# Autodesk Inventor assembly: LockMechanism_v3
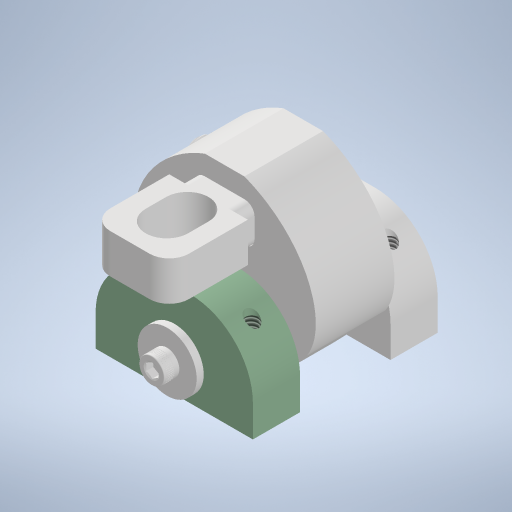
[picture p0: Inventor's stored thumbnail of the model, 512x512]
Saved by Autodesk Inventor 2023 (Build 270158000, 158)
## iProperties
Created: 2023-01-14
Part Number: LockMechanism_v3
Document SubType Name: Assembly
Designer: Hayden Swanson
Author: Hayden Swanson
## Documents named in this file (8)
- C:\Users\Hayden Swanson\UNLAssemblyProject\Hardware\ETL\Module Assembly\WAM_v3\LockMechanism_v3.iam
- C:\Users\Hayden Swanson\UNLAssemblyProject\Hardware\ETL\Module Assembly\WAM_v3\cam3.ipt
- C:\Users\Hayden Swanson\UNLAssemblyProject\Hardware\ETL\Module Assembly\WAM_v3\Connecting Rod.ipt
- C:\Users\Hayden Swanson\UNLAssemblyProject\Hardware\ETL\Module Assembly\WAM_v3\94051A206_Titanium Washer.ipt
- C:\Users\Hayden Swanson\UNLAssemblyProject\Hardware\ETL\Module Assembly\WAM_v3\91251A094_Black-Oxide Alloy Steel Socket Head Screw.ipt
- C:\Users\Hayden Swanson\UNLAssemblyProject\Hardware\ETL\Module Assembly\WAM_v3\key.ipt
- C:\Users\Hayden Swanson\UNLAssemblyProject\Hardware\ETL\Module Assembly\WAM_v3\91375A773_Alloy Steel Cup-Point Set Screw.ipt
- C:\Users\Hayden Swanson\UNLAssemblyProject\Hardware\ETL\Module Assembly\WAM_v3\Lock Base3.ipt
## Components (10 placed, 7 different names)
1. cam3:1 — Mate:2, Mate:3, Mate:4, Mate:5, Mate:6
2. Connecting Rod:1 — Mate:5, Mate:7, Mate:8, Mate:11, Mate:14
3. 94051A206_Titanium Washer:1 — Mate:12, Mate:13, Mate:14, Mate:15, Mate:18
4. 94051A206_Titanium Washer:2 — Mate:9, Mate:10, Mate:11, Mate:16, Mate:17
5. 91251A094_Black-Oxide Alloy Steel Socket Head Screw:1 — Mate:15, Mate:18
6. 91251A094_Black-Oxide Alloy Steel Socket Head Screw:2 — Mate:16, Mate:17
7. key:1 — Mate:2, Mate:3, Mate:4
8. 91375A773_Alloy Steel Cup-Point Set Screw:1 — Mate:6
9. Lock Base3:1 — Mate:8, Mate:9, Mate:10
10. Lock Base3:2 — Mate:7, Mate:12, Mate:13
## Relationships (17: Mate 17)
- Mate:2: cam3:1 ↔ key:1
- Mate:3: cam3:1 ↔ key:1
- Mate:4: cam3:1 ↔ key:1
- Mate:5: cam3:1 ↔ Connecting Rod:1
- Mate:6: cam3:1 ↔ 91375A773_Alloy Steel Cup-Point Set Screw:1
- Mate:7: Connecting Rod:1 ↔ Lock Base3:2
- Mate:8: Connecting Rod:1 ↔ Lock Base3:1
- Mate:9: 94051A206_Titanium Washer:2 ↔ Lock Base3:1
- Mate:10: 94051A206_Titanium Washer:2 ↔ Lock Base3:1
- Mate:11: Connecting Rod:1 ↔ 94051A206_Titanium Washer:2
- Mate:12: 94051A206_Titanium Washer:1 ↔ Lock Base3:2
- Mate:13: 94051A206_Titanium Washer:1 ↔ Lock Base3:2
- Mate:14: Connecting Rod:1 ↔ 94051A206_Titanium Washer:1
- Mate:15: 94051A206_Titanium Washer:1 ↔ 91251A094_Black-Oxide Alloy Steel Socket Head Screw:1
- Mate:16: 94051A206_Titanium Washer:2 ↔ 91251A094_Black-Oxide Alloy Steel Socket Head Screw:2
- Mate:17: 94051A206_Titanium Washer:2 ↔ 91251A094_Black-Oxide Alloy Steel Socket Head Screw:2
- Mate:18: 94051A206_Titanium Washer:1 ↔ 91251A094_Black-Oxide Alloy Steel Socket Head Screw:1
